# Autodesk Inventor assembly: Enclosure
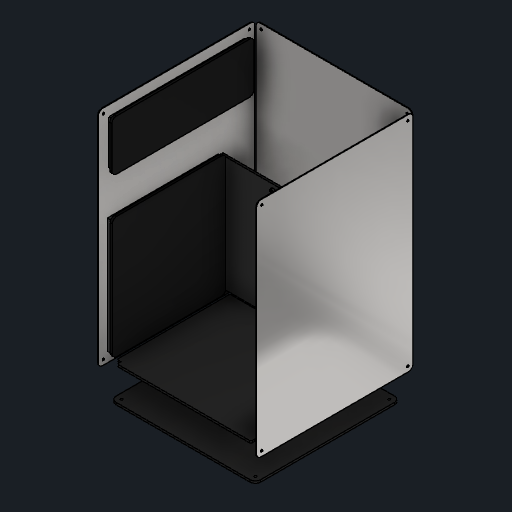
[picture p0: Inventor's stored thumbnail of the model, 512x512]
Saved by Autodesk Inventor 2026.1 (Build 301233020, 233B)
## iProperties
Created: 2025-05-19
Part Number: Enclosure
Document SubType Name: Assembly
Designer: Joshua Eah
Author: Joshua Eah
## Documents named in this file (7)
- C:\Users\JoshuaEah\Documents\GitHub\Voron-0\CAD\Master Assembly\Panels\Enclosure.iam
- C:\Users\JoshuaEah\Documents\GitHub\Voron-0\CAD\Master Assembly\Panels\Parts\Metal Panels\Side Panel.ipt
- C:\Users\JoshuaEah\Documents\GitHub\Voron-0\CAD\Master Assembly\Panels\Parts\Panels\Inner Lower Panel.ipt
- C:\Users\JoshuaEah\Documents\GitHub\Voron-0\CAD\Master Assembly\Panels\Parts\Panels\Inner Top Panel.ipt
- C:\Users\JoshuaEah\Documents\GitHub\Voron-0\CAD\Master Assembly\Panels\Subassemblies\Opaque Panels.iam
- C:\Users\JoshuaEah\Documents\GitHub\Voron-0\CAD\Master Assembly\Panels\Parts\Insulation\Side Foam.ipt
- C:\Users\JoshuaEah\Documents\GitHub\Voron-0\CAD\Master Assembly\Panels\Parts\Insulation\Side Top Foam.ipt
## Components (12 placed, 6 different names)
1. Side Panel:1
2. Side Panel:2
3. Side Panel:3
4. Inner Lower Panel:1 — Mate:1, Flush:1, Flush:2
5. Inner Top Panel:1 — Mate:3, Flush:5, Flush:6
6. Inner Lower Panel:2 — Mate:2, Flush:3, Flush:4
7. Inner Top Panel:2 — Mate:4, Flush:7, Flush:8
8. Opaque Panels:1 [sub-assembly]
9. Side Foam:1 — Mate:1, Flush:1, Flush:2
10. Side Foam:2 — Mate:2, Flush:3, Flush:4
11. Side Top Foam:1 — Mate:3, Flush:5, Flush:6
12. Side Top Foam:2 — Mate:4, Flush:7, Flush:8
## Relationships (12: Flush 8, Mate 4)
- Mate:1: Inner Lower Panel:1 ↔ Side Foam:1
- Flush:1 (2 mm): Inner Lower Panel:1 ↔ Side Foam:1
- Flush:2 (4.5 mm): Inner Lower Panel:1 ↔ Side Foam:1
- Mate:2: Inner Lower Panel:2 ↔ Side Foam:2
- Flush:3 (2 mm): Inner Lower Panel:2 ↔ Side Foam:2
- Flush:4 (4.5 mm): Inner Lower Panel:2 ↔ Side Foam:2
- Mate:3: Inner Top Panel:1 ↔ Side Top Foam:1
- Flush:5 (4.5 mm): Inner Top Panel:1 ↔ Side Top Foam:1
- Flush:6 (4.5 mm): Inner Top Panel:1 ↔ Side Top Foam:1
- Mate:4: Inner Top Panel:2 ↔ Side Top Foam:2
- Flush:7 (4.5 mm): Inner Top Panel:2 ↔ Side Top Foam:2
- Flush:8 (4.5 mm): Inner Top Panel:2 ↔ Side Top Foam:2
